# Autodesk Inventor assembly: rear_bumper_brace
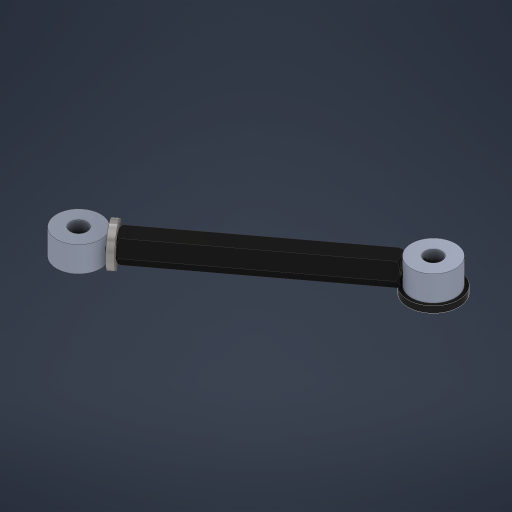
[picture p0: Inventor's stored thumbnail of the model, 512x512]
Saved by Autodesk Inventor 2024 (Build 280153000, 153)
## iProperties
Created: 2024-02-11
Part Number: rear_bumper_brace
Document SubType Name: Assembly
Designer: Averey Ku
Author: Averey Ku
## Documents named in this file (7)
- D:\vex_robotics\hardware\cad\vroomba_v0.1\chassis\rear_bumper_brace.iam
- D:\vex_robotics\hardware\cad\VEX-CAD-Inventor-1.41\Motion\Shaft LS\Shaft Collar ipts\Shaft Collar No Screw.ipt
- D:\vex_robotics\hardware\cad\VEX-CAD-Inventor-1.41\Motion\Spacers\Washer Delrin\DWasher .500 OD x .062500.ipt
- D:\vex_robotics\hardware\cad\VEX-CAD-Inventor-1.41\Motion\Spacers\Washer Steel\SWasher .375 OD x .062500.ipt
- D:\vex_robotics\hardware\cad\VEX-CAD-Inventor-1.41\Motion\Spacers\Washer Steel.ipt
- D:\vex_robotics\hardware\cad\VEX-CAD-Inventor-1.41\Structure\Standoff\Standoff 2.00.ipt
- D:\vex_robotics\hardware\cad\VEX-CAD-Inventor-1.41\Structure\Standoff.ipt
## Components (5 placed, 4 different names)
1. Shaft Collar No Screw:1 — Insert:1, Insert:2
2. Shaft Collar No Screw:2 — Insert:1, Insert:3
3. DWasher .500 OD x .062500:1 — Insert:2
4. SWasher .375 OD x .062500:1 — Insert:3, Insert:4
5. Standoff 2.00:1 — Insert:4
## Relationships (5: Insert 4, Mate 1)
- [Mate]: Shaft Collar No Screw:1 ↔ Shaft Collar No Screw:2
- Insert:1 (52.5 mm): Shaft Collar No Screw:1 ↔ Shaft Collar No Screw:2
- Insert:2: Shaft Collar No Screw:1 ↔ DWasher .500 OD x .062500:1
- Insert:3: Shaft Collar No Screw:2 ↔ SWasher .375 OD x .062500:1
- Insert:4: SWasher .375 OD x .062500:1 ↔ Standoff 2.00:1
